# Autodesk Inventor assembly: Kauri Assembly
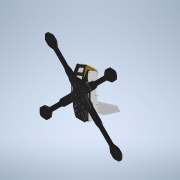
[picture p0: Inventor's stored thumbnail of the model, 180x180]
Saved by Autodesk Inventor 2020 (Build 240168000, 168)
## iProperties
Created: 2022-08-09
Part Number: Kauri Assembly
Document SubType Name: Assembly
Designer: Steven
Author: Steven
## Documents named in this file (12)
- Y:\FPV drone stuff\0 Street League\Frames\PB-Kauri-X\3D prints\35 mm canopy\work in progress prints\Canopy mods\Kauri Assembly.iam
- Y:\FPV drone stuff\0 Street League\Frames\PB-Kauri-X\Kauri bottom plate.ipt
- Y:\FPV drone stuff\0 Street League\Frames\PB-Kauri-X\Kauri mid plate v2.ipt
- Y:\FPV drone stuff\0 Street League\Frames\experimental-quad-frames\modified Kauri arms\disc aero arms\Kauri arm disc aero.ipt
- Y:\FPV drone stuff\0 Street League\Frames\experimental-quad-frames\modified Kauri arms\disc aero arms\Kauri arm long disc aero.ipt
- Y:\FPV drone stuff\0 Street League\Frames\PB-Kauri-X\3D prints\35 mm canopy\KauriFrontLink 35mm.ipt
- Y:\FPV drone stuff\0 Street League\Frames\PB-Kauri-X\Kauri side plate.ipt
- Y:\FPV drone stuff\0 Street League\Frames\PB-Kauri-X\3D prints\35 mm canopy\KauriCanopy Pb.ipt
- Y:\FPV drone stuff\0 Street League\Frames\PB-Kauri-X\3D prints\35 mm canopy\Spoiler v13 35mm.ipt
- Y:\FPV drone stuff\0 Street League\Frames\PB-Kauri-X\3D prints\35 mm canopy\Tall KauriSpoilerFin V2.ipt
- Y:\FPV drone stuff\0 Street League\Frames\PB-Kauri-X\3D prints\35 mm canopy\work in progress prints\Canopy mods\KauriRearLink high rise 35mm no brass insert.ipt
- Y:\FPV drone stuff\0 Street League\Frames\PB-Kauri-X\3D prints\35 mm canopy\work in progress prints\Canopy mods\side skert high rise rear link.ipt
## Components (15 placed, 11 different names)
1. Kauri bottom plate:1 — Mate:1, Mate:2, Flush:1, Flush:2, Flush:3, Mate:3, Mate:4, Mate:5, Mate:6, Mate:7, Mate:8, Mate:9, Mate:10, Mate:11, Mate:12, Mate:38, Mate:39, Mate:40
2. Kauri mid plate v2:1 — Mate:13, Mate:14, Mate:15, Mate:16, Mate:17, Mate:18
3. Kauri arm disc aero:1 — Mate:1, Mate:3, Mate:5
4. Kauri arm disc aero:2 — Mate:2, Mate:4, Mate:6, Mate:14, Mate:15
5. Kauri arm long disc aero:1 — Mate:8, Mate:10, Mate:11
6. Kauri arm long disc aero:2 — Mate:7, Mate:9, Mate:12, Mate:13
7. KauriFrontLink 35mm:1 — Mate:16, Mate:17, Mate:18, Mate:22, Mate:23, Mate:24, Mate:25
8. Kauri side plate:1 — Mate:23, Mate:25, Mate:28, Mate:37, Mate:42, Mate:43, Mate:44
9. Kauri side plate:2 — Mate:22, Mate:24, Mate:29, Mate:30, Mate:31, Mate:32, Mate:33, Mate:41, Flush:4
10. KauriCanopy Pb:1 — Mate:28, Mate:29, Mate:30, Mate:37
11. Spoiler v13 35mm:1 — Mate:31, Mate:32, Mate:33, Mate:34, Mate:35, Mate:36
12. Tall KauriSpoilerFin V2:1 — Mate:34, Mate:35, Mate:36
13. KauriRearLink high rise 35mm no brass insert:1 — Mate:38, Mate:39, Mate:40, Mate:41
14. side skert high rise rear link:1 — Flush:4
15. side skert high rise rear link:2 — Mate:42, Mate:43, Mate:44
## Relationships (43: Mate 39, Flush 4)
- Mate:1: Kauri bottom plate:1 ↔ Kauri arm disc aero:1
- Mate:2: Kauri bottom plate:1 ↔ Kauri arm disc aero:2
- Flush:1: Kauri bottom plate:1
- Flush:2: Kauri bottom plate:1
- Flush:3: Kauri bottom plate:1
- Mate:3: Kauri bottom plate:1 ↔ Kauri arm disc aero:1
- Mate:4: Kauri bottom plate:1 ↔ Kauri arm disc aero:2
- Mate:5: Kauri bottom plate:1 ↔ Kauri arm disc aero:1
- Mate:6: Kauri bottom plate:1 ↔ Kauri arm disc aero:2
- Mate:7: Kauri bottom plate:1 ↔ Kauri arm long disc aero:2
- Mate:8: Kauri bottom plate:1 ↔ Kauri arm long disc aero:1
- Mate:9: Kauri bottom plate:1 ↔ Kauri arm long disc aero:2
- Mate:10: Kauri bottom plate:1 ↔ Kauri arm long disc aero:1
- Mate:11: Kauri bottom plate:1 ↔ Kauri arm long disc aero:1
- Mate:12: Kauri bottom plate:1 ↔ Kauri arm long disc aero:2
- Mate:13: Kauri mid plate v2:1 ↔ Kauri arm long disc aero:2
- Mate:14: Kauri mid plate v2:1 ↔ Kauri arm disc aero:2
- Mate:15: Kauri mid plate v2:1 ↔ Kauri arm disc aero:2
- Mate:16: Kauri mid plate v2:1 ↔ KauriFrontLink 35mm:1
- Mate:17: Kauri mid plate v2:1 ↔ KauriFrontLink 35mm:1
- Mate:18: Kauri mid plate v2:1 ↔ KauriFrontLink 35mm:1
- Mate:22: KauriFrontLink 35mm:1 ↔ Kauri side plate:2
- Mate:23: KauriFrontLink 35mm:1 ↔ Kauri side plate:1
- Mate:24: KauriFrontLink 35mm:1 ↔ Kauri side plate:2
- Mate:25: KauriFrontLink 35mm:1 ↔ Kauri side plate:1
- Mate:28: Kauri side plate:1 ↔ KauriCanopy Pb:1
- Mate:29: Kauri side plate:2 ↔ KauriCanopy Pb:1
- Mate:30: Kauri side plate:2 ↔ KauriCanopy Pb:1
- Mate:31: Kauri side plate:2 ↔ Spoiler v13 35mm:1
- Mate:32: Kauri side plate:2 ↔ Spoiler v13 35mm:1
- Mate:33: Kauri side plate:2 ↔ Spoiler v13 35mm:1
- Mate:34: Spoiler v13 35mm:1 ↔ Tall KauriSpoilerFin V2:1
- Mate:35: Spoiler v13 35mm:1 ↔ Tall KauriSpoilerFin V2:1
- Mate:36: Spoiler v13 35mm:1 ↔ Tall KauriSpoilerFin V2:1
- Mate:37: Kauri side plate:1 ↔ KauriCanopy Pb:1
- Mate:38: Kauri bottom plate:1 ↔ KauriRearLink high rise 35mm no brass insert:1
- Mate:39: Kauri bottom plate:1 ↔ KauriRearLink high rise 35mm no brass insert:1
- Mate:40: Kauri bottom plate:1 ↔ KauriRearLink high rise 35mm no brass insert:1
- Mate:41: Kauri side plate:2 ↔ KauriRearLink high rise 35mm no brass insert:1
- Flush:4: Kauri side plate:2 ↔ side skert high rise rear link:1
- Mate:42: Kauri side plate:1 ↔ side skert high rise rear link:2
- Mate:43: Kauri side plate:1 ↔ side skert high rise rear link:2
- Mate:44: Kauri side plate:1 ↔ side skert high rise rear link:2
